# Autodesk Inventor assembly: Gripper
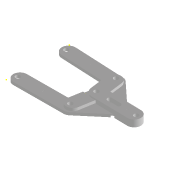
[picture p0: Inventor's stored thumbnail of the model, 180x180]
Saved by Autodesk Inventor 2021 (Build 250183000, 183)
## iProperties
Created: 2022-10-02
Part Number: Gripper
Document SubType Name: Assembly
Designer: brian
Author: brian
## Documents named in this file (4)
- G:\Mi unidad\Universidad\Control\Robotica\Laboratorio\Proyecto\Gripper.iam
- G:\Mi unidad\Universidad\Control\Robotica\Laboratorio\Proyecto\GripP1.ipt
- G:\Mi unidad\Universidad\Control\Robotica\Laboratorio\Proyecto\GripP3.ipt
- G:\Mi unidad\Universidad\Control\Robotica\Laboratorio\Proyecto\GripP4.ipt
## Components (5 placed, 3 different names)
1. GripP1:1 — Rotational:5, Rotational:7
2. GripP3:1 — Rotational:3, Rotational:5, Rotational:6
3. GripP1:2 — Rotational:4, Rotational:7, Tangent:1
4. GripP3:2 — Rotational:3, Rotational:4
5. GripP4:2 — Rotational:6, Tangent:1
## Relationships (6: RevoluteJoint 5, Tangent 1)
- Rotational:3 [RevoluteJoint]: GripP3:1 ↔ GripP3:2
- Rotational:4 [RevoluteJoint]: GripP1:2 ↔ GripP3:2
- Rotational:5 [RevoluteJoint]: GripP1:1 ↔ GripP3:1
- Rotational:6 [RevoluteJoint]: GripP3:1 ↔ GripP4:2
- Rotational:7 [RevoluteJoint]: GripP1:1 ↔ GripP1:2
- Tangent:1: GripP1:2 ↔ GripP4:2
